# Autodesk Inventor assembly: FINALassembly
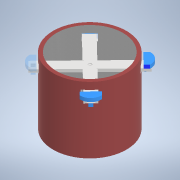
[picture p0: Inventor's stored thumbnail of the model, 180x180]
Saved by Autodesk Inventor 2022 (Build 260153000, 153)
## iProperties
Created: 2021-10-14
Part Number: FINALassembly
Document SubType Name: Assembly
Designer: Nikita
Author: Nikita
## Documents named in this file (3)
- C:\Users\Никита\Documents\FINALassembly.iam
- C:\Users\Никита\Documents\bridgeAssembly.iam
- C:\Users\Никита\Documents\vedro.ipt
## Components (2 placed, 2 different names)
1. bridgeAssembly:1 [sub-assembly] — Mate:1
2. vedro:1 — Mate:1
## Relationships (1: Mate 1)
- Mate:1: bridgeAssembly:1 ↔ vedro:1
